# Autodesk Inventor assembly: 49-0005
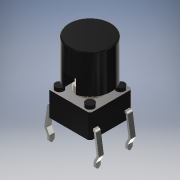
[picture p0: Inventor's stored thumbnail of the model, 180x180]
Saved by Autodesk Inventor 2018 (Build 220112000, 112)
## iProperties
Created: 2019-09-25
Part Number: 49-0005
Document SubType Name: Assembly
Designer: Bradley
Author: Bradley
## Documents named in this file (3)
- C:\Users\Bradley\Documents\GitHub\Resources\SupplierDocuments\49 - Electromechanical\49-0005\49-0005.iam
- C:\Users\Bradley\Documents\GitHub\Resources\SupplierDocuments\49 - Electromechanical\49-0005\49-0005.ipt
- C:\Users\Bradley\Documents\GitHub\Resources\SupplierDocuments\48 - Hardware\48-0077\48-0077.ipt
## Components (2 placed, 2 different names)
1. 49-0005:1 — Mate:1, Flush:1, Flush:2
2. 48-0077:1 — Mate:1, Flush:1, Flush:2
## Relationships (3: Flush 2, Mate 1)
- Mate:1: 49-0005:1 ↔ 48-0077:1
- Flush:1: 49-0005:1 ↔ 48-0077:1
- Flush:2: 49-0005:1 ↔ 48-0077:1
